# Autodesk Inventor assembly: door hinge for arms
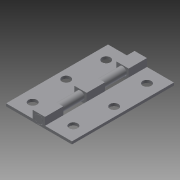
[picture p0: Inventor's stored thumbnail of the model, 180x180]
Saved by Autodesk Inventor 2015 (Build 190159000, 159)
## iProperties
Created: 2015-02-03
Part Number: door hinge for arms
Document SubType Name: Assembly
Designer: szymsea16
Author: szymsea16
## Documents named in this file (4)
- \\lhssvr02\Homedirs\Robotics Club\CAD Model 2015\Box Beam Drive Base\door hinge for arms.iam
- \\lhssvr02\Homedirs\Robotics Club\CAD Model 2015\Box Beam Drive Base\pin for door hinge.ipt
- \\lhssvr02\Homedirs\Robotics Club\CAD Model 2015\Box Beam Drive Base\door hinge for conveyor.ipt
- \\lhssvr02\Homedirs\Robotics Club\CAD Model 2015\Box Beam Drive Base\door hinge for conveyor part 2.ipt
## Components (3 placed, 3 different names)
1. pin for door hinge:1 — Mate:1, Mate:2, Flush:1
2. door hinge for conveyor:1 — Mate:2, Flush:1, Flush:2, Flush:3
3. door hinge for conveyor part 2:1 — Mate:1, Flush:2, Flush:3
## Relationships (5: Flush 3, Mate 2)
- Mate:1: pin for door hinge:1 ↔ door hinge for conveyor part 2:1
- Mate:2: pin for door hinge:1 ↔ door hinge for conveyor:1
- Flush:1: pin for door hinge:1 ↔ door hinge for conveyor:1
- Flush:2: door hinge for conveyor:1 ↔ door hinge for conveyor part 2:1
- Flush:3: door hinge for conveyor:1 ↔ door hinge for conveyor part 2:1
